# Autodesk Inventor assembly: Front_Frame_Fixer
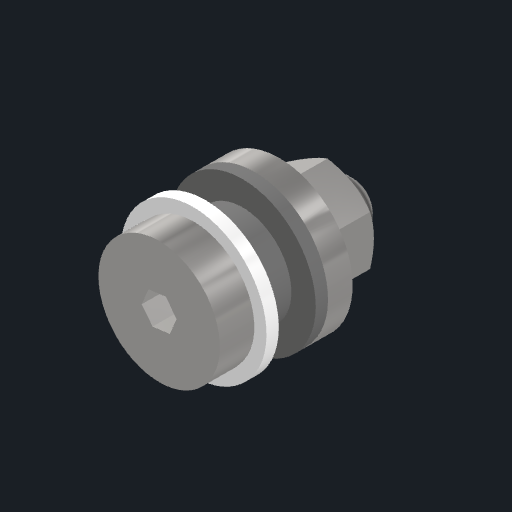
[picture p0: Inventor's stored thumbnail of the model, 512x512]
Saved by Autodesk Inventor 2024.3 (Build 283343000, 343)
## iProperties
Created: 2024-01-28
Part Number: Front_Frame_Fixer
Document SubType Name: Assembly
Designer: 김대겸
Author: 김대겸
## Documents named in this file (6)
- C:\Users\ASUS\Desktop\test\v4_Frame_2025\Front_Frame_Fixer_v2.iam
- C:\Users\ASUS\Desktop\test\v1_Frame\MISUMI\C-WSSA12-4-2.ipt
- C:\Users\ASUS\Desktop\test\v1_Frame\MISUMI\80F-0603.ipt
- C:\Users\ASUS\Desktop\test\v1_Frame\MISUMI\SLBNR4.ipt
- C:\Users\ASUS\Desktop\test\v1_Frame\MISUMI\TT-0612-10.ipt
- C:\Users\ASUS\Desktop\test\v2_Frame\MISUMI\DBSY4-5-8.ipt
## Components (5 placed, 5 different names)
1. C-WSSA12-4-2:1
2. 80F-0603:1 — 삽입:1
3. SLBNR4:1
4. TT-0612-10:1 — 삽입:1, 삽입:2
5. DBSY4-5-8:1 — 삽입:2
## Relationships (2: Insert 2)
- 삽입:1 [Insert]: 80F-0603:1 ↔ TT-0612-10:1
- 삽입:2 [Insert]: TT-0612-10:1 ↔ DBSY4-5-8:1
